# Autodesk Inventor assembly: 組合1
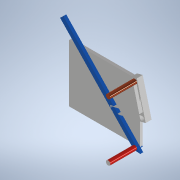
[picture p0: Inventor's stored thumbnail of the model, 180x180]
Saved by Autodesk Inventor 2022 (Build 260153000, 153)
## iProperties
Created: 2023-03-09
Part Number: 組合1
Document SubType Name: Assembly
Designer: JOU
Author: JOU
## Documents named in this file (4)
- C:\Users\JOU\Desktop\實務\組合1.iam
- C:\Users\JOU\Desktop\實務\零件3.ipt
- C:\Users\JOU\Desktop\實務\零件2.ipt
- C:\Users\JOU\Desktop\實務\零件4.ipt
## Components (4 placed, 3 different names)
1. 零件3:1 — 貼合:1, 齊平:1, 貼合:4, 齊平:3
2. 零件4:1 — 貼合:1, 齊平:1, 貼合:2, 齊平:2
3. 零件4:2 — 貼合:2, 齊平:2, 貼合:3
4. 零件2:1 — 貼合:3, 貼合:4, 齊平:3
## Relationships (7: Mate 4, Flush 3)
- 貼合:1 [Mate]: 零件3:1 ↔ 零件4:1
- 齊平:1 [Flush]: 零件3:1 ↔ 零件4:1
- 貼合:2 [Mate]: 零件4:1 ↔ 零件4:2
- 齊平:2 [Flush]: 零件4:1 ↔ 零件4:2
- 貼合:3 [Mate]: 零件4:2 ↔ 零件2:1
- 貼合:4 [Mate]: 零件3:1 ↔ 零件2:1
- 齊平:3 [Flush]: 零件3:1 ↔ 零件2:1
